# Autodesk Inventor assembly: Palma
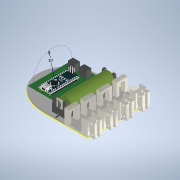
[picture p0: Inventor's stored thumbnail of the model, 180x180]
Saved by Autodesk Inventor 2020.4 (Build 244396010, 396A)
## iProperties
Created: 2021-08-20
Part Number: Palma
Document SubType Name: Assembly
Designer: chalo
Author: chalo
## Documents named in this file (8)
- C:\Users\chalo\OneDrive\Documents\GitHub\Interfaces-Biomedicas-2021\Gonzalo Palarea\Inventor\_completa\Palma.iam
- C:\Users\chalo\OneDrive\Documents\GitHub\Interfaces-Biomedicas-2021\Gonzalo Palarea\Inventor\tipo2\Palma.ipt
- C:\Users\chalo\OneDrive\Documents\GitHub\Interfaces-Biomedicas-2021\Gonzalo Palarea\Inventor\referencias\18650.ipt
- C:\Users\chalo\OneDrive\Documents\GitHub\Interfaces-Biomedicas-2021\Gonzalo Palarea\Inventor\referencias\Battery Holder 18650_COMF_BHC-18650-1A.ipt
- C:\Users\chalo\OneDrive\Documents\GitHub\Interfaces-Biomedicas-2021\Gonzalo Palarea\Inventor\tipo2\Metacarpo.ipt
- C:\Users\chalo\OneDrive\Documents\GitHub\Interfaces-Biomedicas-2021\Gonzalo Palarea\Inventor\tipo2\Falange_media_distal.ipt
- C:\Users\chalo\OneDrive\Documents\GitHub\Interfaces-Biomedicas-2021\Gonzalo Palarea\Inventor\referencias\PCB_Prueba.iam
- C:\Users\chalo\OneDrive\Documents\GitHub\Interfaces-Biomedicas-2021\Gonzalo Palarea\Inventor\Ensamblaje_Final\ipts\Base_final.ipt
## Components (13 placed, 7 different names)
1. Palma:1 — Mate:5, Angle:1, Flush:1, Flush:2, Flush:3, Flush:4, Flush:5, Flush:6, Flush:7, Flush:8, Flush:9, Flush:10
2. 18650:2 — Mate:4, Tangent:1, Tangent:2
3. Battery Holder 18650_COMF_BHC-18650-1A:1 — Mate:4, Tangent:1, Mate:5, Tangent:2, Angle:1
4. Metacarpo:1 — Insert:2
5. Falange_media_distal:1 — Insert:2
6. PCB_Prueba:1 [sub-assembly]
7. Base_final:1 — Flush:4, Flush:9, Flush:10
8. Base_final:2 — Flush:3, Flush:8, Mate:7
9. Base_final:3 — Flush:2, Flush:7, Mate:6, Mate:7
10. Base_final:4 — Flush:1, Flush:5, Flush:6, Mate:6
11. Battery Holder 18650_COMF_BHC-18650-1A:2
12. 18650:3
13. Base_final:5
## Relationships (18: Flush 10, Mate 4, Tangent 2, Angle 1, Insert 1)
- Mate:4: 18650:2 ↔ Battery Holder 18650_COMF_BHC-18650-1A:1
- Tangent:1: 18650:2 ↔ Battery Holder 18650_COMF_BHC-18650-1A:1
- Mate:5: Palma:1 ↔ Battery Holder 18650_COMF_BHC-18650-1A:1
- Tangent:2 (1 mm): 18650:2 ↔ Battery Holder 18650_COMF_BHC-18650-1A:1
- Angle:1 (0 deg): Palma:1 ↔ Battery Holder 18650_COMF_BHC-18650-1A:1
- Insert:2: Metacarpo:1 ↔ Falange_media_distal:1
- Flush:1: Palma:1 ↔ Base_final:4
- Flush:2: Palma:1 ↔ Base_final:3
- Flush:3: Palma:1 ↔ Base_final:2
- Flush:4: Palma:1 ↔ Base_final:1
- Flush:5: Palma:1 ↔ Base_final:4
- Flush:6: Palma:1 ↔ Base_final:4
- Flush:7: Palma:1 ↔ Base_final:3
- Flush:8: Palma:1 ↔ Base_final:2
- Flush:9: Palma:1 ↔ Base_final:1
- Flush:10: Palma:1 ↔ Base_final:1
- Mate:6 (7 mm): Base_final:3 ↔ Base_final:4
- Mate:7 (7 mm): Base_final:2 ↔ Base_final:3
